# Autodesk Inventor assembly: 000200
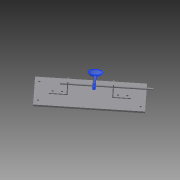
[picture p0: Inventor's stored thumbnail of the model, 180x180]
Saved by Autodesk Inventor 2015 (Build 190159000, 159)
## iProperties
Created: 2015-05-27
Part Number: 000200
Document SubType Name: Assembly
Designer: Wesley
Author: Wesley
## Documents named in this file (5)
- C:\Users\Wesley\Documents\GitHub\EngineeringFinal\Engineering\Engineering Documentation\CADS\0002__\000200.iam
- C:\Users\Wesley\Documents\GitHub\EngineeringFinal\Engineering\Engineering Documentation\CADS\0002__\000201.ipt
- C:\Users\Wesley\Documents\GitHub\EngineeringFinal\Engineering\Engineering Documentation\CADS\0002__\000204.ipt
- C:\Users\Wesley\Documents\GitHub\EngineeringFinal\Engineering\Engineering Documentation\CADS\0002__\000203.ipt
- C:\Users\Wesley\Documents\GitHub\EngineeringFinal\Engineering\Engineering Documentation\CADS\0002__\000205.ipt
## Components (5 placed, 4 different names)
1. 000201:1 — Mate:1, Mate:2, Mate:3, Mate:4, Mate:5, Mate:6
2. 000204:1 — Mate:1, Mate:2, Mate:3, Mate:7
3. 000204:2 — Mate:4, Mate:5, Mate:6
4. 000203:1 — Mate:7, Mate:8
5. 000205:1 — Mate:8
## Relationships (8: Mate 8)
- Mate:1: 000201:1 ↔ 000204:1
- Mate:2: 000201:1 ↔ 000204:1
- Mate:3: 000201:1 ↔ 000204:1
- Mate:4: 000201:1 ↔ 000204:2
- Mate:5: 000201:1 ↔ 000204:2
- Mate:6: 000201:1 ↔ 000204:2
- Mate:7: 000204:1 ↔ 000203:1
- Mate:8: 000203:1 ↔ 000205:1
